# Autodesk Inventor assembly: Sub system 2 Assembly
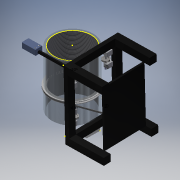
[picture p0: Inventor's stored thumbnail of the model, 180x180]
Saved by Autodesk Inventor 2019 (Build 230136000, 136)
## iProperties
Created: 2020-02-19
Part Number: Sub system 2 Assembly
Document SubType Name: Assembly
Designer: Adityan Matthew
Author: Adityan Matthew
## Documents named in this file (9)
- D:\Sub system 2 Assembly.iam
- D:\Eexp.1.ipt
- D:\Eexp.4.ipt
- D:\Assembly5.iam
- D:\water dispenser.ipt
- D:\tray.ipt
- D:\Motor DC.ipt
- D:\DC motor base.ipt
- D:\Sub system 2 Assembly\Design Accelerator\V-Belt transmission5.iam
## Components (11 placed, 8 different names)
1. Eexp.1:1
2. Eexp.4:1 — Mate:1, Rotational:1, Rotational:2
3. Assembly5:1 [sub-assembly]
4. Assembly5:2 [sub-assembly] — Mate:1
5. Assembly5:3 [sub-assembly]
6. Assembly5:4 [sub-assembly]
7. water dispenser:1 — Rotational:1, Rotational:2
8. tray:1
9. Motor DC:1 — Cylindrical:1
10. DC motor base:1 — Cylindrical:1
11. V-Belt transmission:1 [sub-assembly]
## Relationships (4: RevoluteJoint 2, Mate 1, CylindricalJoint 1)
- Mate:1: Eexp.4:1 ↔ Assembly5:2
- Rotational:1 [RevoluteJoint] (-100 mm): Eexp.4:1 ↔ water dispenser:1
- Rotational:2 [RevoluteJoint] (-100 mm): Eexp.4:1 ↔ water dispenser:1
- Cylindrical:1: Motor DC:1 ↔ DC motor base:1
